# Autodesk Inventor assembly: CL7-200
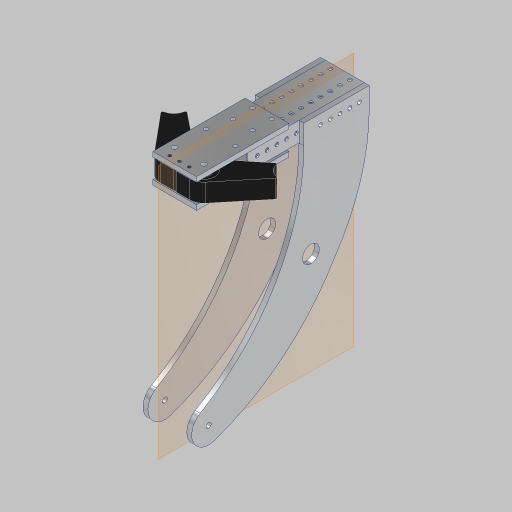
[picture p0: Inventor's stored thumbnail of the model, 512x512]
Saved by Autodesk Inventor 2023.5 (Build 275446000, 446)
## iProperties
Created: 2025-03-17
Part Number: CL7-200
Document SubType Name: Assembly
Designer: dlangdon
Author: dlangdon
## Documents named in this file (6)
- C:\Users\slick\OneDrive\Desktop\2025-ReefScape---CAD\Climber\CL7\CL7-200.iam
- C:\Users\slick\OneDrive\Desktop\2025-ReefScape---CAD\Climber\CL7\CL7-005.ipt
- C:\Users\slick\OneDrive\Desktop\2025-ReefScape---CAD\Climber\CL7\CL7-004.ipt
- C:\Users\slick\OneDrive\Desktop\2025-ReefScape---CAD\Climber\CL7\CL7-005aa.ipt
- C:\Users\slick\OneDrive\Desktop\2025-ReefScape---CAD\Climber\CL7\CL7-006.ipt
- C:\Users\slick\OneDrive\Desktop\2025-ReefScape---CAD\Climber\CL7\CL7-008.ipt
## Components (7 placed, 5 different names)
1. CL7-005:1 — Mate:4, Mate:5, Mate:6, Mate:7, Mate:8, Mate:9, Insert:1, Insert:2
2. CL7-004:1 — Mate:5, Flush:1
3. CL7-004:2 — Mate:4, Mate:6, Flush:1
4. CL7-005aa:1 — Mate:7, Mate:8, Mate:9
5. CL7-006:1 — Insert:1, Insert:2, Insert:3, Insert:4, Insert:5, Insert:6
6. CL7-008:1 — Insert:3, Insert:4, Symmetry:1
7. CL7-008:2 — Insert:5, Insert:6, Symmetry:1
## Relationships (14: Mate 6, Insert 6, Flush 1, Symmetry 1)
- Mate:4: CL7-005:1 ↔ CL7-004:2
- Mate:5: CL7-005:1 ↔ CL7-004:1
- Mate:6 (0.7937 mm): CL7-005:1 ↔ CL7-004:2
- Flush:1: CL7-004:1 ↔ CL7-004:2
- Mate:7: CL7-005:1 ↔ CL7-005aa:1
- Mate:8: CL7-005:1 ↔ CL7-005aa:1
- Mate:9 (25.4 mm): CL7-005:1 ↔ CL7-005aa:1
- Insert:1: CL7-005:1 ↔ CL7-006:1
- Insert:2: CL7-005:1 ↔ CL7-006:1
- Insert:3: CL7-006:1 ↔ CL7-008:1
- Insert:4: CL7-006:1 ↔ CL7-008:1
- Insert:5: CL7-006:1 ↔ CL7-008:2
- Insert:6: CL7-006:1 ↔ CL7-008:2
- Symmetry:1: CL7-008:1 ↔ CL7-008:2
